# Autodesk Inventor assembly: 01 Gripper_System
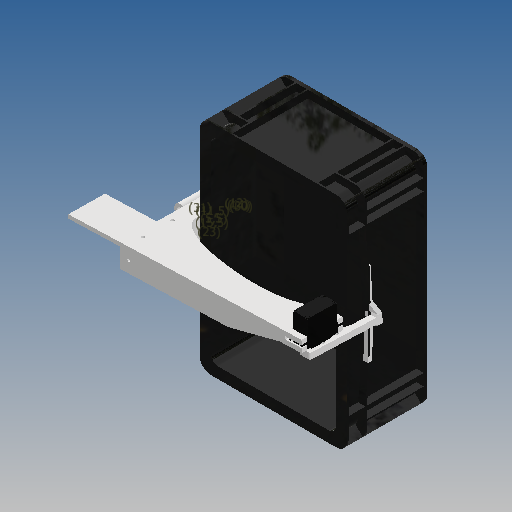
[picture p0: Inventor's stored thumbnail of the model, 512x512]
Saved by Autodesk Inventor 2026.2 (Build 302298000, 298)
## iProperties
Created: 2025-12-10
Part Number: 01 Gripper_System
Document SubType Name: Assembly
Designer: Schally
Author: Schally
## Documents named in this file (6)
- E:\06 Carologistics\02 Zeichnungen Greifer System\Gripper alt\01 Gripper_System.iam
- E:\06 Carologistics\02 Zeichnungen Greifer System\Gripper alt\01-02 Servo_Gripper.iam
- E:\06 Carologistics\02 Zeichnungen Greifer System\Gripper alt\00 Zeichnung Box.ipt
- E:\06 Carologistics\02 Zeichnungen Greifer System\Gripper alt\01-01 Gripper_Basis_Neu.ipt
- E:\06 Carologistics\02 Zeichnungen Greifer System\Gripper alt\01-03 Zangensystem Gripper unten.iam
- E:\06 Carologistics\02 Zeichnungen Greifer System\Gripper alt\01-05 Absicherung Richtung Kugellager.ipt
## Components (5 placed, 5 different names)
1. 00 Zeichnung Box:1
2. 01-01 Gripper_Basis_Neu:1 — Einfügen:3, Einfügen:6, Passend:1
3. 01-02 Servo_Gripper:1 [sub-assembly] — Einfügen:3
4. 01-05 Absicherung Richtung Kugellager:1 — Einfügen:6, Passend:2
5. 01-03 Zangensystem Gripper unten:2 [sub-assembly] — Passend:1, Passend:2
## Relationships (4: Insert 2, Mate 2)
- Einfügen:3 [Insert] (0.5 mm): 01-01 Gripper_Basis_Neu:1 ↔ 01-02 Servo_Gripper:1
- Einfügen:6 [Insert]: 01-01 Gripper_Basis_Neu:1 ↔ 01-05 Absicherung Richtung Kugellager:1
- Passend:1 [Mate]: 01-01 Gripper_Basis_Neu:1 ↔ 01-03 Zangensystem Gripper unten:2
- Passend:2 [Mate]: 01-05 Absicherung Richtung Kugellager:1 ↔ 01-03 Zangensystem Gripper unten:2
